# Autodesk Inventor assembly: Assembly_Matchboxscope_injectionmolded
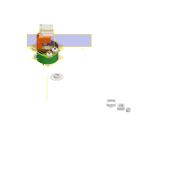
[picture p0: Inventor's stored thumbnail of the model, 180x180]
Saved by Autodesk Inventor 2022 (Build 260153000, 153)
## iProperties
Created: 2023-04-12
Part Number: Assembly_Matchboxscope_injectionmolded
Document SubType Name: Assembly
Designer: diederichbenedict
Author: diederichbenedict
## Documents named in this file (18)
- C:\Users\diederichbenedict\Dropbox\Dokumente\Promotion\PROJECTS\Matchboxscope\INVENTOR\RELEASE\InjectionMolded\Assembly_Matchboxscope_injectionmolded.iam
- C:\Users\diederichbenedict\Dropbox\Dokumente\Promotion\PROJECTS\Matchboxscope\INVENTOR\RELEASE\InjectionMolded\IM_Matchboxscope_base.ipt
- C:\Users\diederichbenedict\Dropbox\Dokumente\Promotion\PROJECTS\Matchboxscope\INVENTOR\RELEASE\InjectionMolded\IM_Matchboxscope_plate.ipt
- C:\Users\diederichbenedict\Dropbox\Dokumente\Promotion\PROJECTS\Matchboxscope\INVENTOR\RELEASE\InjectionMolded\IM_Lensholder.ipt
- C:\Users\diederichbenedict\Dropbox\Dokumente\Promotion\PROJECTS\Matchboxscope\INVENTOR\RELEASE\InjectionMolded\IM_Periscope.ipt
- C:\Users\diederichbenedict\Dropbox\Dokumente\Promotion\PROJECTS\Matchboxscope\INVENTOR\RELEASE\InjectionMolded\IM_ledholder.ipt
- C:\Users\diederichbenedict\Dropbox\Dokumente\Promotion\PROJECTS\Matchboxscope\INVENTOR\RELEASE\InjectionMolded\Anglerfish_Cameraspacer.ipt
- C:\Users\diederichbenedict\Dropbox\Dokumente\Promotion\PROJECTS\Matchboxscope\INVENTOR\RELEASE\InjectionMolded\00_CCTV_M12_VCM_large.ipt
- C:\Users\diederichbenedict\Dropbox\Dokumente\Promotion\PROJECTS\Matchboxscope\INVENTOR\RELEASE\InjectionMolded\IM_Lensholder_M12.ipt
- C:\Users\diederichbenedict\Dropbox\Dokumente\Promotion\PROJECTS\Matchboxscope\INVENTOR\RELEASE\InjectionMolded\Matchboxscope_M12_Lensadapter_v0.ipt
- C:\Users\diederichbenedict\Dropbox\Dokumente\Promotion\PROJECTS\Matchboxscope\INVENTOR\RELEASE\InjectionMolded\00_Turningscrew.ipt
- C:\Users\diederichbenedict\Documents\Inventor\Content Center Files\R2022\de-DE\DIN 912\DIN 912 - M3 x 0.5 x 25 x 18.ipt
- C:\Users\diederichbenedict\Documents\Inventor\Content Center Files\R2022\de-DE\DIN 912\DIN 912 - M3 x 0.5 x 10 x 8.75.ipt
- C:\Users\diederichbenedict\Dropbox\Dokumente\Promotion\PROJECTS\Matchboxscope\INVENTOR\RELEASE\InjectionMolded\00_LED_lamp.ipt
- C:\Users\diederichbenedict\Dropbox\Dokumente\Promotion\PROJECTS\Matchboxscope\INVENTOR\RELEASE\InjectionMolded\IM_Matchboxscope_lightdiffusor_ring.ipt
- C:\Users\diederichbenedict\Dropbox\Dokumente\Promotion\PROJECTS\Matchboxscope\INVENTOR\RELEASE\InjectionMolded\00_Neopixel_4x4_Matrix.ipt
- C:\Users\diederichbenedict\Dropbox\Dokumente\Promotion\PROJECTS\Matchboxscope\INVENTOR\RELEASE\InjectionMolded\IM_ledmatrix_holder.ipt
- C:\Users\diederichbenedict\Dropbox\Dokumente\Promotion\PROJECTS\Matchboxscope\INVENTOR\RELEASE\InjectionMolded\IM_ledmatrix_diffuser.ipt
## Components (24 placed, 17 different names)
1. IM_Matchboxscope_base:1 — Fluchtend:1, Einfügen:15, Passend:3
2. IM_Matchboxscope_plate:1 — Einfügen:10
3. IM_Lensholder:1 — Fluchtend:1, Einfügen:8
4. IM_Periscope:1
5. IM_ledholder:1 — Einfügen:9, Einfügen:14, Winkel:3, Passend:4, Passend:5, Passend:6, Fluchtend:2
6. Anglerfish_Cameraspacer:1
7. 00_CCTV_M12_VCM_large:1 — Passend:2, Winkel:2
8. IM_Lensholder_M12:1 — Passend:2, Winkel:2
9. Matchboxscope_M12_Lensadapter_v0:1
10. 00_Turningscrew:1
11. DIN 912 - ersetzt durch DIN EN ISO 4762 M3 x 25:1
12. DIN 912 - ersetzt durch DIN EN ISO 4762 M3 x 25:2
13. DIN 912 - ersetzt durch DIN EN ISO 4762 M3 x 25:3
14. DIN 912 - ersetzt durch DIN EN ISO 4762 M3 x 10:1 — Einfügen:10
15. DIN 912 - ersetzt durch DIN EN ISO 4762 M3 x 10:2 — Einfügen:9
16. DIN 912 - ersetzt durch DIN EN ISO 4762 M3 x 10:3 — Einfügen:8
17. 00_Turningscrew:2
18. 00_Turningscrew:3
19. 00_LED_lamp:1 — Einfügen:14
20. IM_Matchboxscope_lightdiffusor_ring:1
21. IM_Matchboxscope_plate:2 — Einfügen:15, Passend:3, Winkel:3, Passend:4, Passend:5, Passend:6, Fluchtend:2, Passend:7, Passend:8, Winkel:4, Fluchtend:3, Fluchtend:4
22. 00_Neopixel_4x4_Matrix:1 — Passend:7, Passend:8, Winkel:4
23. IM_ledmatrix_holder:1 — Fluchtend:3, Fluchtend:4, Fluchtend:5, Fluchtend:6
24. IM_ledmatrix_diffuser:1 — Fluchtend:5, Fluchtend:6
## Relationships (23: Insert 7, Mate 7, Flush 6, Angle 3)
- [Insert]: IM_Matchboxscope_base:1 ↔ IM_Matchboxscope_plate:1
- [Insert]: IM_Matchboxscope_base:1 ↔ IM_Matchboxscope_plate:1
- Fluchtend:1 [Flush]: IM_Matchboxscope_base:1 ↔ IM_Lensholder:1
- Passend:2 [Mate]: 00_CCTV_M12_VCM_large:1 ↔ IM_Lensholder_M12:1
- Winkel:2 [Angle] (45 deg): 00_CCTV_M12_VCM_large:1 ↔ IM_Lensholder_M12:1
- Einfügen:8 [Insert]: IM_Lensholder:1 ↔ DIN 912 - ersetzt durch DIN EN ISO 4762 M3 x 10:3
- Einfügen:9 [Insert]: IM_ledholder:1 ↔ DIN 912 - ersetzt durch DIN EN ISO 4762 M3 x 10:2
- Einfügen:10 [Insert] (-4 mm): IM_Matchboxscope_plate:1 ↔ DIN 912 - ersetzt durch DIN EN ISO 4762 M3 x 10:1
- Einfügen:14 [Insert]: IM_ledholder:1 ↔ 00_LED_lamp:1
- Einfügen:15 [Insert] (5 mm): IM_Matchboxscope_base:1 ↔ IM_Matchboxscope_plate:2
- Passend:3 [Mate]: IM_Matchboxscope_base:1 ↔ IM_Matchboxscope_plate:2
- Winkel:3 [Angle] (0 deg): IM_ledholder:1 ↔ IM_Matchboxscope_plate:2
- Passend:4 [Mate]: IM_ledholder:1 ↔ IM_Matchboxscope_plate:2
- Passend:5 [Mate]: IM_ledholder:1 ↔ IM_Matchboxscope_plate:2
- Passend:6 [Mate]: IM_ledholder:1 ↔ IM_Matchboxscope_plate:2
- Fluchtend:2 [Flush]: IM_ledholder:1 ↔ IM_Matchboxscope_plate:2
- Passend:7 [Mate] (50 mm): IM_Matchboxscope_plate:2 ↔ 00_Neopixel_4x4_Matrix:1
- Passend:8 [Mate]: IM_Matchboxscope_plate:2 ↔ 00_Neopixel_4x4_Matrix:1
- Winkel:4 [Angle] (180 deg): IM_Matchboxscope_plate:2 ↔ 00_Neopixel_4x4_Matrix:1
- Fluchtend:3 [Flush]: IM_Matchboxscope_plate:2 ↔ IM_ledmatrix_holder:1
- Fluchtend:4 [Flush]: IM_Matchboxscope_plate:2 ↔ IM_ledmatrix_holder:1
- Fluchtend:5 [Flush]: IM_ledmatrix_holder:1 ↔ IM_ledmatrix_diffuser:1
- Fluchtend:6 [Flush]: IM_ledmatrix_holder:1 ↔ IM_ledmatrix_diffuser:1
